# Autodesk Inventor assembly: slider for beam diameter
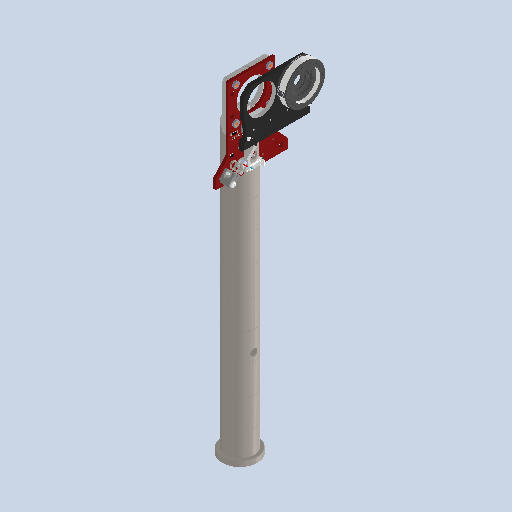
[picture p0: Inventor's stored thumbnail of the model, 512x512]
Saved by Autodesk Inventor 2026.1 (Build 301233000, 233)
## iProperties
Created: 2025-06-02
Part Number: slider for beam diameter
Document SubType Name: Assembly
Designer: Julian
Author: Julian
## Documents named in this file (7)
- C:\Users\user\Desktop\setup_inventor_2025\slider beam diameter\slider for beam diameter.iam
- C:\Users\user\Desktop\setup_inventor_2025\slider beam diameter\ELL6.ipt
- C:\Users\user\Desktop\setup_inventor_2025\slider beam diameter\Newport-M-PS-4-1.ipt
- C:\Users\user\Desktop\setup_inventor_2025\slider beam diameter\Newport-M-PS-6E-.ipt
- C:\Users\user\Desktop\setup_inventor_2025\slider beam diameter\RS4_M.ipt
- C:\Users\user\Desktop\setup_inventor_2025\slider beam diameter\ELLA1-Step.ipt
- C:\Users\user\Desktop\setup_inventor_2025\slider beam diameter\SM1D12D.ipt
## Components (6 placed, 6 different names)
1. ELL6:1 — Passend:1, Passend:2, Passend:3, Passend:10, Passend:11
2. Newport-M-PS-4-1:1 — Passend:4, Passend:5
3. Newport-M-PS-6E-:1 — Passend:4, Passend:5, Passend:6, Passend:7
4. RS4_M:1 — Passend:6, Passend:7, Passend:8, Passend:9
5. ELLA1-Step:1 — Passend:1, Passend:2, Passend:3, Passend:8, Passend:9
6. SM1D12D:1 — Passend:10, Passend:11
## Relationships (11: Mate 11)
- Passend:1 [Mate]: ELL6:1 ↔ ELLA1-Step:1
- Passend:2 [Mate]: ELL6:1 ↔ ELLA1-Step:1
- Passend:3 [Mate]: ELL6:1 ↔ ELLA1-Step:1
- Passend:4 [Mate]: Newport-M-PS-4-1:1 ↔ Newport-M-PS-6E-:1
- Passend:5 [Mate]: Newport-M-PS-4-1:1 ↔ Newport-M-PS-6E-:1
- Passend:6 [Mate]: Newport-M-PS-6E-:1 ↔ RS4_M:1
- Passend:7 [Mate]: Newport-M-PS-6E-:1 ↔ RS4_M:1
- Passend:8 [Mate]: RS4_M:1 ↔ ELLA1-Step:1
- Passend:9 [Mate]: RS4_M:1 ↔ ELLA1-Step:1
- Passend:10 [Mate]: ELL6:1 ↔ SM1D12D:1
- Passend:11 [Mate]: ELL6:1 ↔ SM1D12D:1
